# Autodesk Inventor assembly: Tall Cylinder & Cap
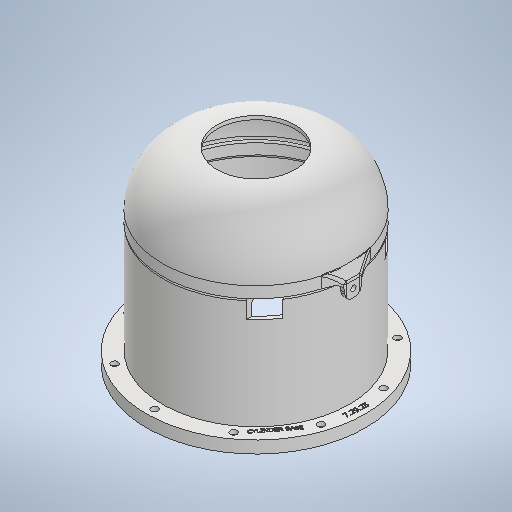
[picture p0: Inventor's stored thumbnail of the model, 512x512]
Saved by Autodesk Inventor 2025 (Build 290162000, 162)
## iProperties
Created: 2025-07-29
Part Number: Tall Cylinder & Cap
Document SubType Name: Assembly
Designer: mumin
Author: mumin
## Documents named in this file (3)
- C:\GitHub\In-situ-monitoring-of-powder-bed-fusion-additive-manufacturing\system_development\Orichalcum\v0.3\Tall Cylinder & Cap.iam
- C:\GitHub\In-situ-monitoring-of-powder-bed-fusion-additive-manufacturing\system_development\Orichalcum\v0.3\Cylinder Housing_base.ipt
- C:\GitHub\In-situ-monitoring-of-powder-bed-fusion-additive-manufacturing\system_development\Orichalcum\v0.3\Cylinder Housing_cap_2.ipt
## Components (2 placed, 2 different names)
1. Cylinder Housing_base:1 — Mate:1, Mate:2
2. Cylinder Housing_cap_2:1 — Mate:1, Mate:2
## Relationships (2: Mate 2)
- Mate:1: Cylinder Housing_base:1 ↔ Cylinder Housing_cap_2:1
- Mate:2: Cylinder Housing_base:1 ↔ Cylinder Housing_cap_2:1
